# Autodesk Inventor assembly: Assembly_Axiotech_Eypiece
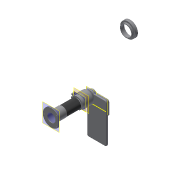
[picture p0: Inventor's stored thumbnail of the model, 180x180]
Saved by Autodesk Inventor 2019 (Build 230136000, 136)
## iProperties
Created: 2019-06-02
Part Number: Assembly_Axiotech_Eypiece
Document SubType Name: Assembly
Designer: diederichbenedict
Author: diederichbenedict
## Documents named in this file (6)
- C:\Users\diederichbenedict\Dropbox\Dokumente\Promotion\PROJECTS\STORMoChip\INVENTOR\Nanoscopy-on-a-cheap\Assembly_Axiotech_Eypiece.iam
- C:\Users\diederichbenedict\Dropbox\Dokumente\Promotion\PROJECTS\STORMoChip\INVENTOR\Nanoscopy-on-a-cheap\00_Zeiss_Axiotech_Eyepiecemount.ipt
- C:\Users\diederichbenedict\Dropbox\Dokumente\Promotion\PROJECTS\STORMoChip\INVENTOR\Nanoscopy-on-a-cheap\10_Zeiss_Axiotech_Eypiecemount_Adapter.ipt
- C:\Users\diederichbenedict\Dropbox\Dokumente\Promotion\PROJECTS\STORMoChip\INVENTOR\Nanoscopy-on-a-cheap\SM30L20-Step.ipt
- C:\Users\diederichbenedict\Dropbox\Dokumente\Promotion\PROJECTS\STORMoChip\INVENTOR\Nanoscopy-on-a-cheap\Assembly_cellphoneadapter.iam
- C:\Users\diederichbenedict\Dropbox\Dokumente\Promotion\PROJECTS\STORMoChip\INVENTOR\Nanoscopy-on-a-cheap\101_Illumination_Adapter_Axiotech_COOLled.ipt
## Components (5 placed, 5 different names)
1. 00_Zeiss_Axiotech_Eyepiecemount:1 — Flush:1, Flush:2
2. 10_Zeiss_Axiotech_Eypiecemount_Adapter:1 — Flush:1, Flush:2, Insert:1
3. SM30L20-Step:1 — Insert:1, Insert:2
4. Assembly_cellphoneadapter:1 [sub-assembly] — Insert:2
5. 101_Illumination_Adapter_Axiotech_COOLled:1
## Relationships (4: Flush 2, Insert 2)
- Flush:1: 00_Zeiss_Axiotech_Eyepiecemount:1 ↔ 10_Zeiss_Axiotech_Eypiecemount_Adapter:1
- Flush:2: 00_Zeiss_Axiotech_Eyepiecemount:1 ↔ 10_Zeiss_Axiotech_Eypiecemount_Adapter:1
- Insert:1: 10_Zeiss_Axiotech_Eypiecemount_Adapter:1 ↔ SM30L20-Step:1
- Insert:2: SM30L20-Step:1 ↔ Assembly_cellphoneadapter:1
